# Autodesk Inventor assembly: recuperation
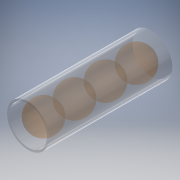
[picture p0: Inventor's stored thumbnail of the model, 180x180]
Saved by Autodesk Inventor 2017 (Build 210142000, 142)
## iProperties
Created: 2018-03-31
Part Number: recuperation
Document SubType Name: Assembly
Designer: franc
Author: franc
## Documents named in this file (3)
- C:\Users\franc\Desktop\EsialRobotik\Mecanique\2018\robot\traitement-eau\recuperation.iam
- C:\Users\franc\Desktop\EsialRobotik\Mecanique\2018\robot\traitement-eau\cylindre-stockage.ipt
- C:\Users\franc\Desktop\EsialRobotik\Mecanique\2018\robot\traitement-eau\eau.ipt
## Components (5 placed, 2 different names)
1. cylindre-stockage:1 — Placage:1, Placage:2, Tangente:1, Placage:3, Placage:4
2. eau:1 — Placage:1, Tangente:1, Tangente:2
3. eau:2 — Placage:2, Tangente:2, Tangente:3
4. eau:3 — Placage:3, Tangente:3, Tangente:4
5. eau:4 — Placage:4, Tangente:4
## Relationships (8: Mate 4, Tangent 4)
- Placage:1 [Mate]: cylindre-stockage:1 ↔ eau:1
- Placage:2 [Mate]: cylindre-stockage:1 ↔ eau:2
- Tangente:1: cylindre-stockage:1 ↔ eau:1
- Tangente:2: eau:1 ↔ eau:2
- Placage:3 [Mate]: cylindre-stockage:1 ↔ eau:3
- Tangente:3: eau:2 ↔ eau:3
- Placage:4 [Mate]: cylindre-stockage:1 ↔ eau:4
- Tangente:4: eau:3 ↔ eau:4
